# Autodesk Inventor assembly: v5马达+四方轴套+螺丝
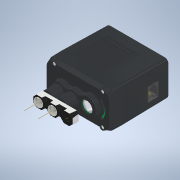
[picture p0: Inventor's stored thumbnail of the model, 180x180]
Saved by Autodesk Inventor 2020 (Build 240168000, 168)
## iProperties
Created: 2019-06-01
Part Number: v5马达+四方轴套+螺丝
Document SubType Name: Assembly
Designer: hp
Author: hp
## Documents named in this file (4)
- C:\Users\hp\Documents\Vault\ncrCadLib\V5主控系统\v5马达+四方轴套+螺丝.iam
- C:\Users\hp\Documents\Vault\ncrCadLib\V5主控系统\V5_Smart_Motor_276-4840.iam
- C:\Users\hp\Documents\Vault\ncrCadLib\轴相关\细轴配套\零件\细轴四方轴承.ipt
- C:\Users\hp\Documents\Vault\ncrCadLib\螺丝螺帽\Screw 8-32 x 0.500'' 三号.ipt
## Components (4 placed, 3 different names)
1. V5_Smart_Motor_276-4840:1 [sub-assembly] — 配合:1, 配合:2, 配合:3
2. 细轴四方轴承:1 — 配合:1, 配合:2, 配合:3, 配合:4, 配合:5, 配合:6, 配合:7
3. Screw 8-32 x 0.500'' 三号:1 — 配合:4, 配合:7
4. Screw 8-32 x 0.500'' 三号:2 — 配合:5, 配合:6
## Relationships (7: Mate 7)
- 配合:1 [Mate]: V5_Smart_Motor_276-4840:1 ↔ 细轴四方轴承:1
- 配合:2 [Mate]: V5_Smart_Motor_276-4840:1 ↔ 细轴四方轴承:1
- 配合:3 [Mate] (1.5748 mm): V5_Smart_Motor_276-4840:1 ↔ 细轴四方轴承:1
- 配合:4 [Mate]: 细轴四方轴承:1 ↔ Screw 8-32 x 0.500'' 三号:1
- 配合:5 [Mate]: 细轴四方轴承:1 ↔ Screw 8-32 x 0.500'' 三号:2
- 配合:6 [Mate]: 细轴四方轴承:1 ↔ Screw 8-32 x 0.500'' 三号:2
- 配合:7 [Mate]: 细轴四方轴承:1 ↔ Screw 8-32 x 0.500'' 三号:1
